# Autodesk Inventor assembly: Bartender Robot Asm
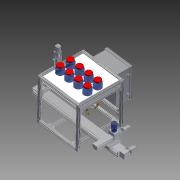
[picture p0: Inventor's stored thumbnail of the model, 180x180]
Saved by Autodesk Inventor 2011 (Build 150239000, 239)
## iProperties
Created: 2013-10-23
Part Number: Bartender Robot Asm
Document SubType Name: Assembly
Designer: Devon
Author: Devon
## Documents named in this file (31)
- C:\Users\Devon\Dropbox\ELEC 4497 - Senior Design\Design\Bartender Robot Asm.iam
- C:\Users\Devon\Dropbox\ELEC 4497 - Senior Design\Design\1.5 in. aluminum extrusion\Imported Components\47065T210\Part32.ipt
- C:\Users\Devon\Dropbox\ELEC 4497 - Senior Design\Design\1.5 in. aluminum extrusion\Imported Components\47065T210\Part34.ipt
- C:\Users\Devon\Dropbox\ELEC 4497 - Senior Design\Design\extrusion fittings\Imported Components\1.5in 3 sided fastener\Assembly5.iam
- C:\Users\Devon\Dropbox\ELEC 4497 - Senior Design\Design\extrusion fittings\Imported Components\1.5in 3 sided fastener\Assembly1.iam
- C:\Users\Devon\Dropbox\ELEC 4497 - Senior Design\Design\1.5 in. aluminum extrusion\Imported Components\47065T210\Part10.ipt
- C:\Users\Devon\Dropbox\ELEC 4497 - Senior Design\Design\extrusion fittings\Imported Components\1.5in 2 sided fastener\Assembly2.iam
- C:\Users\Devon\Dropbox\ELEC 4497 - Senior Design\Design\Enclosure\Imported Components\Enclosure\Assembly3.iam
- C:\Users\Devon\Dropbox\ELEC 4497 - Senior Design\Design\340mm KR linear actuator\PARTserver64610126with cover\KR45H 10A + 340L0 - 10A0(0-0).iam
- C:\Users\Devon\Dropbox\ELEC 4497 - Senior Design\Design\Liquid Vessel\Vessel.ipt
- C:\Users\Devon\Dropbox\ELEC 4497 - Senior Design\Design\1.5 in. aluminum extrusion\Imported Components\47065T210\Part3.ipt
- C:\Users\Devon\Dropbox\ELEC 4497 - Senior Design\Design\lexan panels\vessel support bottom.ipt
- C:\Users\Devon\Dropbox\ELEC 4497 - Senior Design\Design\lexan panels\vessel support top.ipt
- C:\Users\Devon\Dropbox\ELEC 4497 - Senior Design\Design\1.5 in. aluminum extrusion\Imported Components\47065T210\Part5.ipt
- C:\Users\Devon\Dropbox\ELEC 4497 - Senior Design\Design\machined mounts\xy axis mount.ipt
- C:\Users\Devon\Dropbox\ELEC 4497 - Senior Design\Design\machined mounts\glass socket.ipt
- C:\Users\Devon\Dropbox\ELEC 4497 - Senior Design\Design\glass\glass.ipt
- C:\Users\Devon\Dropbox\ELEC 4497 - Senior Design\Design\1.5 in. aluminum extrusion\7in.ipt
- C:\Users\Devon\Dropbox\ELEC 4497 - Senior Design\Design\servo motor\nema 23 frame size servo.ipt
- C:\Users\Devon\Dropbox\ELEC 4497 - Senior Design\Design\980mm KR linear actuator\NEMA23 frame size\GL20N-142-SW-EH--C-N-N-Y_(804U1).iam
- C:\Users\Devon\Dropbox\ELEC 4497 - Senior Design\Design\flow\flow meter solenoid asm.iam
- C:\Users\Devon\Dropbox\ELEC 4497 - Senior Design\Design\lexan panels\mixer support.ipt
- C:\Users\Devon\Dropbox\ELEC 4497 - Senior Design\Design\1.5 in. aluminum extrusion\5.094in.ipt
- C:\Users\Devon\Dropbox\ELEC 4497 - Senior Design\Design\Imported Components\5537T510\Part4.ipt
- C:\Users\Devon\Dropbox\ELEC 4497 - Senior Design\Design\Imported Components\5537T510\Part6.ipt
- C:\Users\Devon\Dropbox\ELEC 4497 - Senior Design\Design\Imported Components\5537T510\Part8.ipt
- C:\Users\Devon\Dropbox\ELEC 4497 - Senior Design\Design\Imported Components\5537T510\Part10.ipt
- C:\Users\Devon\Dropbox\ELEC 4497 - Senior Design\Design\Imported Components\5537T510\Part12.ipt
- C:\Users\Devon\Dropbox\ELEC 4497 - Senior Design\Design\Liquid Vessel\cap.ipt
- C:\Users\Devon\Dropbox\ELEC 4497 - Senior Design\Design\lexan panels\splash guard.ipt
- C:\Users\Devon\Dropbox\ELEC 4497 - Senior Design\Design\1.5 in. aluminum extrusion\Imported Components\47065T210\Part4.ipt
## Components (93 placed, 28 different names)
1. Part32:2 — Mate:10, Flush:19, Flush:20, Mate:15, Flush:27, Flush:28, Mate:30, Mate:103, Flush:92, Mate:106
2. Part32:3 — Mate:5, Flush:9, Flush:10, Mate:13, Flush:23, Flush:24, Flush:36, Flush:42, Mate:52, Mate:89, Flush:85, Mate:91, Flush:86, Mate:98, Flush:89, Mate:99, Flush:90, Flush:102, Mate:130, Flush:103, Mate:132, Flush:104
3. Part32:4 — Mate:2, Flush:3, Flush:4, Mate:9, Flush:17, Flush:18, Mate:125, Flush:111
4. Part32:5 — Mate:8, Flush:15, Flush:16, Mate:14, Flush:25, Flush:26, Flush:43, Mate:93, Flush:87, Mate:96, Flush:88, Mate:107, Mate:110
5. Part32:6 — Mate:1, Flush:1, Flush:2, Flush:3, Mate:4, Flush:7, Flush:8, Flush:55
6. Part32:7 — Mate:6, Flush:11, Flush:12, Mate:7, Flush:13, Flush:14, Mate:19, Flush:35
7. Part34:1 — Mate:3, Flush:5, Flush:6, Mate:16, Flush:29, Flush:30, Mate:29, Mate:101, Flush:91, Mate:112, Mate:126, Mate:128, Mate:134, Flush:105, Mate:136, Flush:106
8. Assembly5:1 [sub-assembly] — Mate:1, Flush:1, Flush:2, Mate:2, Flush:4, Mate:3, Flush:5, Flush:6
9. Assembly1:1 [sub-assembly] — Mate:4, Flush:7, Flush:8, Mate:5, Flush:9, Flush:10, Mate:6, Flush:11, Flush:12, Mate:21
10. Assembly1:2 [sub-assembly] — Mate:7, Flush:13, Flush:14, Mate:8, Flush:15, Flush:16, Mate:11, Flush:22
11. Assembly1:3 [sub-assembly] — Mate:9, Flush:17, Flush:18, Mate:10, Flush:19, Flush:20, Mate:12, Flush:21
12. Part10:1 — Mate:11, Mate:12, Flush:21, Flush:22, Mate:56
13. Part10:2 — Mate:17, Flush:31, Flush:32, Mate:73, Flush:77, Mate:75, Flush:78, Mate:86, Mate:87, Flush:84
14. Part10:3 — Mate:18, Flush:33, Flush:34, Mate:22, Flush:38, Mate:23, Flush:39, Mate:78, Mate:79, Flush:80, Mate:81, Flush:81, Mate:83, Flush:82
15. Assembly2:1 [sub-assembly] — Mate:16, Flush:29, Flush:30
16. Assembly2:2 [sub-assembly] — Mate:13, Flush:23, Flush:24, Mate:18, Flush:33, Flush:34, Mate:20
17. Assembly2:3 [sub-assembly] — Mate:14, Flush:25, Flush:26
18. Assembly2:4 [sub-assembly] — Mate:15, Flush:27, Flush:28, Mate:17, Flush:31, Flush:32
19. Assembly3:1 [sub-assembly] — Mate:19, Flush:35, Flush:37, Mate:21
20. Part32:8 — Mate:20, Flush:36, Flush:37, Mate:90, Mate:92, Mate:94, Mate:95
21. Part34:2 — Mate:22, Flush:38, Tangent:2, Tangent:5, Mate:46, Mate:82, Mate:84, Mate:85, Flush:83, Mate:88
22. Part34:3 — Mate:23, Flush:39, Tangent:3, Tangent:4, Mate:74, Mate:76, Mate:77, Flush:79, Mate:80
23. KR45H 10A + 340L0 - 10A0(0-0):1 [sub-assembly] — Flush:51, Flush:52, Mate:38, Flush:63, Mate:47, Flush:64, Flush:67, Flush:68, Mate:50
24. Vessel:1 — Insert:10, Mate:61, Mate:124, Insert:16
25. Vessel:2 — Insert:11, Mate:57, Mate:120, Insert:15
26. Part3:2 — Mate:29, Flush:42, Flush:59, Mate:55, Mate:97, Mate:100, Mate:102, Mate:111, Flush:96, Mate:139
27. vessel support bottom:1 — Insert:4, Insert:5, Insert:6, Insert:7, Insert:8, Insert:9, Insert:10, Insert:11, Mate:52, Mate:53, Mate:54, Mate:55, Tangent:6, Tangent:7, Tangent:8, Tangent:9, Tangent:10, Tangent:11, Tangent:12, Tangent:13, Flush:112, Flush:113, Flush:114, Flush:115, Flush:116, Flush:117, Flush:118, Flush:119
28. vessel support top:1 — Flush:55, Flush:59, Mate:56
29. Part5:2 — Mate:30, Flush:43, Mate:53, Mate:54, Mate:104, Mate:105, Flush:93, Mate:108, Flush:94, Mate:109, Flush:95
30. xy axis mount:1 — Flush:63, Mate:47, Flush:64, Mate:48, Flush:65, Flush:66
31. glass socket:1 — Flush:51, Flush:52, Mate:38, Insert:2
32. glass:1 — Insert:2
33. Vessel:3 — Insert:7, Mate:60, Mate:117, Insert:12
34. Vessel:4 — Insert:4, Mate:63, Mate:122, Insert:18
35. Vessel:5 — Insert:8, Mate:62, Mate:123, Insert:17
36. Vessel:6 — Insert:5, Mate:64, Mate:121, Insert:19
37. Vessel:7 — Insert:6, Mate:59, Mate:118, Insert:13
38. Vessel:8 — Insert:9, Mate:58, Mate:119, Insert:14
39. 7in:1 — Mate:65, Mate:67, Mate:69, Flush:71, Flush:72, Mate:114, Flush:101, Flush:108, Flush:109
40. 7in:2 — Mate:68, Mate:70, Flush:73, Flush:74, Mate:115, Flush:98, Mate:137, Mate:138, Flush:107
41. KR45H 10A + 340L0 - 10A0(0-0):2 [sub-assembly] — Flush:61, Flush:62, Mate:49, Flush:110, Mate:139
42. nema 23 frame size servo:1 — Flush:61, Flush:62, Mate:49
43. GL20N-142-SW-EH--C-N-N-Y_(804U1):1 [sub-assembly] — Tangent:2, Tangent:3, Tangent:4, Tangent:5, Mate:46, Mate:48, Flush:65, Flush:66, Flush:69, Flush:70, Mate:140
44. nema 23 frame size servo:2 — Flush:67, Flush:68, Mate:50
45. nema 23 frame size servo:3 — Flush:69, Flush:70, Mate:140
46. flow meter solenoid asm:1 [sub-assembly] — Mate:57, Tangent:6, Flush:119
47. flow meter solenoid asm:2 [sub-assembly] — Mate:63, Tangent:12, Flush:114
48. flow meter solenoid asm:3 [sub-assembly] — Mate:61, Tangent:10, Flush:112
49. flow meter solenoid asm:4 [sub-assembly] — Mate:64, Tangent:13, Flush:115
50. flow meter solenoid asm:5 [sub-assembly] — Mate:62, Tangent:11, Flush:113
51. flow meter solenoid asm:6 [sub-assembly] — Mate:58, Tangent:7, Flush:118
52. flow meter solenoid asm:7 [sub-assembly] — Mate:59, Tangent:8, Flush:117
53. flow meter solenoid asm:8 [sub-assembly] — Mate:60, Tangent:9, Flush:116
54. mixer support:1 — Mate:65, Mate:67, Mate:68, Mate:127
55. Assembly2:5 [sub-assembly] — Mate:69, Flush:71, Flush:72, Mate:72, Flush:75, Flush:76
56. Assembly2:6 [sub-assembly] — Mate:70, Flush:73, Flush:74, Mate:71, Flush:99, Flush:100
57. 5.094in:1 — Mate:71, Mate:72, Flush:75, Flush:76, Flush:99, Flush:100, Mate:127
58. Part4:1 — Mate:73, Mate:74, Flush:77
59. Part6:1 — Mate:77, Mate:78, Flush:79
60. Part6:2 — Mate:81, Mate:82, Flush:81
61. Part6:3 — Mate:75, Mate:76, Flush:78
62. Part6:4 — Mate:89, Mate:90, Flush:85
63. Part6:5 — Mate:93, Mate:94, Flush:87
64. Part6:6 — Mate:101, Mate:102, Flush:91
65. Part6:7 — Mate:87, Mate:88, Flush:84
66. Part6:8 — Mate:91, Mate:92, Flush:86
67. Part6:9 — Mate:85, Mate:86, Flush:83
68. Part6:10 — Mate:103, Mate:104, Flush:92
69. Part6:11 — Mate:105, Mate:106, Flush:93
70. Part6:12 — Mate:99, Mate:100, Flush:90
71. Part6:13 — Mate:97, Mate:98, Flush:89
72. Part6:14 — Mate:107, Mate:108, Flush:94
73. Part6:15 — Mate:83, Mate:84, Flush:82
74. Part6:16 — Mate:95, Mate:96, Flush:88
75. Part6:17 — Mate:79, Mate:80, Flush:80
76. Part8:1 — Mate:109, Mate:110, Flush:95
77. Part10:4 — Mate:111, Mate:112, Flush:96
78. Part12:1 — Mate:114, Flush:101, Flush:108
79. Part12:2 — Mate:115, Flush:98, Mate:138, Flush:107
80. cap:1 — Mate:122, Insert:18
81. cap:2 — Mate:123, Insert:17
82. cap:3 — Mate:124, Insert:16
83. cap:4 — Mate:121, Insert:19
84. cap:5 — Mate:120, Insert:15
85. cap:6 — Mate:119, Insert:14
86. cap:7 — Mate:118, Insert:13
87. cap:8 — Mate:117, Insert:12
88. splash guard:1 — Mate:125, Mate:126, Flush:111
89. Part4:2 — Mate:128, Flush:102, Mate:129, Mate:131, Mate:133, Mate:135, Mate:137, Flush:109, Flush:110
90. Part6:18 — Mate:131, Mate:132, Flush:104
91. Part6:19 — Mate:129, Mate:130, Flush:103
92. Part6:20 — Mate:133, Mate:134, Flush:105
93. Part6:21 — Mate:135, Mate:136, Flush:106
## Relationships (249: Mate 117, Flush 103, Insert 17, Tangent 12)
- Mate:1: Part32:6 ↔ Assembly5:1
- Flush:1 (12.2936 mm): Part32:6 ↔ Assembly5:1
- Flush:2 (12.2936 mm): Part32:6 ↔ Assembly5:1
- Mate:2: Part32:4 ↔ Assembly5:1
- Flush:3: Part32:4 ↔ Part32:6
- Flush:4 (12.2936 mm): Part32:4 ↔ Assembly5:1
- Mate:3: Part34:1 ↔ Assembly5:1
- Flush:5 (12.2936 mm): Part34:1 ↔ Assembly5:1
- Flush:6 (12.2936 mm): Part34:1 ↔ Assembly5:1
- Mate:4: Part32:6 ↔ Assembly1:1
- Flush:7 (12.2936 mm): Part32:6 ↔ Assembly1:1
- Flush:8 (12.2936 mm): Part32:6 ↔ Assembly1:1
- Mate:5: Part32:3 ↔ Assembly1:1
- Flush:9 (12.2936 mm): Part32:3 ↔ Assembly1:1
- Flush:10 (12.2936 mm): Part32:3 ↔ Assembly1:1
- Mate:6: Part32:7 ↔ Assembly1:1
- Flush:11 (12.2936 mm): Part32:7 ↔ Assembly1:1
- Flush:12 (12.2936 mm): Part32:7 ↔ Assembly1:1
- Mate:7: Part32:7 ↔ Assembly1:2
- Flush:13 (-12.2936 mm): Part32:7 ↔ Assembly1:2
- Flush:14 (-12.2936 mm): Part32:7 ↔ Assembly1:2
- Mate:8: Part32:5 ↔ Assembly1:2
- Flush:15 (12.2936 mm): Part32:5 ↔ Assembly1:2
- Flush:16 (12.2936 mm): Part32:5 ↔ Assembly1:2
- Mate:9: Part32:4 ↔ Assembly1:3
- Flush:17 (-12.2936 mm): Part32:4 ↔ Assembly1:3
- Flush:18 (-12.2936 mm): Part32:4 ↔ Assembly1:3
- Mate:10: Part32:2 ↔ Assembly1:3
- Flush:19 (12.2936 mm): Part32:2 ↔ Assembly1:3
- Flush:20 (12.2936 mm): Part32:2 ↔ Assembly1:3
- Mate:11: Assembly1:2 ↔ Part10:1
- Mate:12: Assembly1:3 ↔ Part10:1
- Flush:21 (12.2936 mm): Assembly1:3 ↔ Part10:1
- Flush:22 (12.2936 mm): Assembly1:2 ↔ Part10:1
- Mate:13: Part32:3 ↔ Assembly2:2
- Flush:23 (-12.2936 mm): Part32:3 ↔ Assembly2:2
- Flush:24 (-12.2936 mm): Part32:3 ↔ Assembly2:2
- Mate:14: Part32:5 ↔ Assembly2:3
- Flush:25 (-12.2936 mm): Part32:5 ↔ Assembly2:3
- Flush:26 (-12.2936 mm): Part32:5 ↔ Assembly2:3
- Mate:15: Part32:2 ↔ Assembly2:4
- Flush:27 (-12.2936 mm): Part32:2 ↔ Assembly2:4
- Flush:28 (-12.2936 mm): Part32:2 ↔ Assembly2:4
- Mate:16: Part34:1 ↔ Assembly2:1
- Flush:29 (-12.2936 mm): Part34:1 ↔ Assembly2:1
- Flush:30 (-12.2936 mm): Part34:1 ↔ Assembly2:1
- Mate:17: Part10:2 ↔ Assembly2:4
- Flush:31 (12.2936 mm): Part10:2 ↔ Assembly2:4
- Flush:32 (12.2936 mm): Part10:2 ↔ Assembly2:4
- Mate:18: Part10:3 ↔ Assembly2:2
- Flush:33 (12.2936 mm): Part10:3 ↔ Assembly2:2
- Flush:34 (12.2936 mm): Part10:3 ↔ Assembly2:2
- Mate:19 (12.2936 mm): Part32:7 ↔ Assembly3:1
- Flush:35 (-2.54 mm): Part32:7 ↔ Assembly3:1
- Mate:20: Assembly2:2 ↔ Part32:8
- Flush:36: Part32:3 ↔ Part32:8
- Flush:37 (2.54 mm): Assembly3:1 ↔ Part32:8
- Mate:21 (98.552 mm): Assembly1:1 ↔ Assembly3:1
- Mate:22 (12.2936 mm): Part10:3 ↔ Part34:2
- Flush:38: Part10:3 ↔ Part34:2
- Mate:23 (12.2936 mm): Part10:3 ↔ Part34:3
- Flush:39: Part10:3 ↔ Part34:3
- Mate:29 (12.2936 mm): Part34:1 ↔ Part3:2
- Flush:42: Part32:3 ↔ Part3:2
- Mate:30 (12.2936 mm): Part32:2 ↔ Part5:2
- Flush:43: Part32:5 ↔ Part5:2
- Flush:51: KR45H 10A + 340L0 - 10A0(0-0):1 ↔ glass socket:1
- Flush:52: KR45H 10A + 340L0 - 10A0(0-0):1 ↔ glass socket:1
- Mate:38: KR45H 10A + 340L0 - 10A0(0-0):1 ↔ glass socket:1
- Insert:2: glass socket:1 ↔ glass:1
- Insert:4 (6.35 mm): vessel support bottom:1 ↔ Vessel:4
- Insert:5 (6.35 mm): vessel support bottom:1 ↔ Vessel:6
- Insert:6 (6.35 mm): vessel support bottom:1 ↔ Vessel:7
- Insert:7 (6.35 mm): vessel support bottom:1 ↔ Vessel:3
- Insert:8 (6.35 mm): vessel support bottom:1 ↔ Vessel:5
- Insert:9 (6.35 mm): vessel support bottom:1 ↔ Vessel:8
- Insert:10 (6.35 mm): Vessel:1 ↔ vessel support bottom:1
- Insert:11 (6.35 mm): Vessel:2 ↔ vessel support bottom:1
- Flush:55 (12.2936 mm): Part32:6 ↔ vessel support top:1
- Flush:59: Part3:2 ↔ vessel support top:1
- Flush:61 (2.667 mm): KR45H 10A + 340L0 - 10A0(0-0):2 ↔ nema 23 frame size servo:1
- Flush:62 (1.4224 mm): KR45H 10A + 340L0 - 10A0(0-0):2 ↔ nema 23 frame size servo:1
- Tangent:2: Part34:2 ↔ GL20N-142-SW-EH--C-N-N-Y_(804U1):1
- Tangent:3: Part34:3 ↔ GL20N-142-SW-EH--C-N-N-Y_(804U1):1
- Tangent:4: Part34:3 ↔ GL20N-142-SW-EH--C-N-N-Y_(804U1):1
- Tangent:5: Part34:2 ↔ GL20N-142-SW-EH--C-N-N-Y_(804U1):1
- Mate:46 (12.2936 mm): Part34:2 ↔ GL20N-142-SW-EH--C-N-N-Y_(804U1):1
- Flush:63 (50.2031 mm): KR45H 10A + 340L0 - 10A0(0-0):1 ↔ xy axis mount:1
- Mate:47: KR45H 10A + 340L0 - 10A0(0-0):1 ↔ xy axis mount:1
- Flush:64 (141.8844 mm): KR45H 10A + 340L0 - 10A0(0-0):1 ↔ xy axis mount:1
- Mate:48: xy axis mount:1 ↔ GL20N-142-SW-EH--C-N-N-Y_(804U1):1
- Flush:65: xy axis mount:1 ↔ GL20N-142-SW-EH--C-N-N-Y_(804U1):1
- Flush:66: xy axis mount:1 ↔ GL20N-142-SW-EH--C-N-N-Y_(804U1):1
- Mate:49: KR45H 10A + 340L0 - 10A0(0-0):2 ↔ nema 23 frame size servo:1
- Flush:67 (2.667 mm): KR45H 10A + 340L0 - 10A0(0-0):1 ↔ nema 23 frame size servo:2
- Flush:68 (-1.4224 mm): KR45H 10A + 340L0 - 10A0(0-0):1 ↔ nema 23 frame size servo:2
- Mate:50: KR45H 10A + 340L0 - 10A0(0-0):1 ↔ nema 23 frame size servo:2
- Flush:69 (4.191 mm): GL20N-142-SW-EH--C-N-N-Y_(804U1):1 ↔ nema 23 frame size servo:3
- Flush:70 (4.445 mm): GL20N-142-SW-EH--C-N-N-Y_(804U1):1 ↔ nema 23 frame size servo:3
- Mate:52 (12.2936 mm): Part32:3 ↔ vessel support bottom:1
- Mate:53: vessel support bottom:1 ↔ Part5:2
- Mate:54: vessel support bottom:1 ↔ Part5:2
- Mate:55: Part3:2 ↔ vessel support bottom:1
- Mate:56: Part10:1 ↔ vessel support top:1
- Mate:57: Vessel:2 ↔ flow meter solenoid asm:1
- Tangent:6: vessel support bottom:1 ↔ flow meter solenoid asm:1
- Mate:58: Vessel:8 ↔ flow meter solenoid asm:6
- Tangent:7: vessel support bottom:1 ↔ flow meter solenoid asm:6
- Mate:59: Vessel:7 ↔ flow meter solenoid asm:7
- Tangent:8: vessel support bottom:1 ↔ flow meter solenoid asm:7
- Mate:60: Vessel:3 ↔ flow meter solenoid asm:8
- Tangent:9: vessel support bottom:1 ↔ flow meter solenoid asm:8
- Mate:61: Vessel:1 ↔ flow meter solenoid asm:3
- Tangent:10: vessel support bottom:1 ↔ flow meter solenoid asm:3
- Mate:62: Vessel:5 ↔ flow meter solenoid asm:5
- Tangent:11: vessel support bottom:1 ↔ flow meter solenoid asm:5
- Mate:63: Vessel:4 ↔ flow meter solenoid asm:2
- Tangent:12: vessel support bottom:1 ↔ flow meter solenoid asm:2
- Mate:64: Vessel:6 ↔ flow meter solenoid asm:4
- Tangent:13: vessel support bottom:1 ↔ flow meter solenoid asm:4
- Mate:65: 7in:1 ↔ mixer support:1
- Mate:67: 7in:1 ↔ mixer support:1
- Mate:68: 7in:2 ↔ mixer support:1
- Mate:69: 7in:1 ↔ Assembly2:5
- Flush:71 (-12.2936 mm): 7in:1 ↔ Assembly2:5
- Flush:72 (-12.2936 mm): 7in:1 ↔ Assembly2:5
- Mate:70: 7in:2 ↔ Assembly2:6
- Flush:73 (-12.2936 mm): 7in:2 ↔ Assembly2:6
- Flush:74 (-12.2936 mm): 7in:2 ↔ Assembly2:6
- Mate:71: Assembly2:6 ↔ 5.094in:1
- Mate:72: Assembly2:5 ↔ 5.094in:1
- Flush:75 (12.2936 mm): Assembly2:5 ↔ 5.094in:1
- Flush:76 (12.2936 mm): Assembly2:5 ↔ 5.094in:1
- Mate:73 (12.2936 mm): Part10:2 ↔ Part4:1
- Mate:74 (12.2936 mm): Part34:3 ↔ Part4:1
- Flush:77 (-12.2936 mm): Part10:2 ↔ Part4:1
- Mate:75 (12.2936 mm): Part10:2 ↔ Part6:3
- Mate:76 (12.2936 mm): Part34:3 ↔ Part6:3
- Flush:78 (-12.2936 mm): Part10:2 ↔ Part6:3
- Mate:77 (12.2936 mm): Part34:3 ↔ Part6:1
- Mate:78 (12.2936 mm): Part10:3 ↔ Part6:1
- Flush:79 (-12.2936 mm): Part34:3 ↔ Part6:1
- Mate:79 (12.2936 mm): Part10:3 ↔ Part6:17
- Mate:80 (12.2936 mm): Part34:3 ↔ Part6:17
- Flush:80 (-12.2936 mm): Part10:3 ↔ Part6:17
- Mate:81 (12.2936 mm): Part10:3 ↔ Part6:2
- Mate:82 (12.2936 mm): Part34:2 ↔ Part6:2
- Flush:81 (-12.2936 mm): Part10:3 ↔ Part6:2
- Mate:83 (12.2936 mm): Part10:3 ↔ Part6:15
- Mate:84 (12.2936 mm): Part34:2 ↔ Part6:15
- Flush:82 (-12.2936 mm): Part10:3 ↔ Part6:15
- Mate:85 (12.2936 mm): Part34:2 ↔ Part6:9
- Mate:86 (12.2936 mm): Part10:2 ↔ Part6:9
- Flush:83 (-12.2936 mm): Part34:2 ↔ Part6:9
- Mate:87 (12.2936 mm): Part10:2 ↔ Part6:7
- Mate:88 (12.2936 mm): Part34:2 ↔ Part6:7
- Flush:84 (-12.2936 mm): Part10:2 ↔ Part6:7
- Mate:89 (12.2936 mm): Part32:3 ↔ Part6:4
- Mate:90 (12.2936 mm): Part32:8 ↔ Part6:4
- Flush:85 (-12.2936 mm): Part32:3 ↔ Part6:4
- Mate:91 (12.2936 mm): Part32:3 ↔ Part6:8
- Mate:92 (12.2936 mm): Part32:8 ↔ Part6:8
- Flush:86 (-12.2936 mm): Part32:3 ↔ Part6:8
- Mate:93 (12.2936 mm): Part32:5 ↔ Part6:5
- Mate:94 (12.2936 mm): Part32:8 ↔ Part6:5
- Flush:87 (-12.2936 mm): Part32:5 ↔ Part6:5
- Mate:95 (12.2936 mm): Part32:8 ↔ Part6:16
- Mate:96 (12.2936 mm): Part32:5 ↔ Part6:16
- Flush:88 (-12.2936 mm): Part32:5 ↔ Part6:16
- Mate:97 (12.2936 mm): Part3:2 ↔ Part6:13
- Mate:98 (12.2936 mm): Part32:3 ↔ Part6:13
- Flush:89 (-12.2936 mm): Part32:3 ↔ Part6:13
- Mate:99 (12.2936 mm): Part32:3 ↔ Part6:12
- Mate:100 (12.2936 mm): Part3:2 ↔ Part6:12
- Flush:90 (-12.2936 mm): Part32:3 ↔ Part6:12
- Mate:101 (12.2936 mm): Part34:1 ↔ Part6:6
- Mate:102 (12.2936 mm): Part3:2 ↔ Part6:6
- Flush:91 (-12.2936 mm): Part34:1 ↔ Part6:6
- Mate:103 (12.2936 mm): Part32:2 ↔ Part6:10
- Mate:104 (12.2936 mm): Part5:2 ↔ Part6:10
- Flush:92 (-12.2936 mm): Part32:2 ↔ Part6:10
- Mate:105 (12.2936 mm): Part5:2 ↔ Part6:11
- Mate:106 (12.2936 mm): Part32:2 ↔ Part6:11
- Flush:93 (-12.2936 mm): Part5:2 ↔ Part6:11
- Mate:107 (12.2936 mm): Part32:5 ↔ Part6:14
- Mate:108 (12.2936 mm): Part5:2 ↔ Part6:14
- Flush:94 (-12.2936 mm): Part5:2 ↔ Part6:14
- Mate:109 (12.2936 mm): Part5:2 ↔ Part8:1
- Mate:110 (12.2936 mm): Part32:5 ↔ Part8:1
- Flush:95 (-12.2936 mm): Part5:2 ↔ Part8:1
- Mate:111 (12.2936 mm): Part3:2 ↔ Part10:4
- Mate:112 (12.2936 mm): Part34:1 ↔ Part10:4
- Flush:96 (-12.2936 mm): Part3:2 ↔ Part10:4
- Mate:114 (12.2936 mm): 7in:1 ↔ Part12:1
- Mate:115 (12.2936 mm): 7in:2 ↔ Part12:2
- Flush:98 (-12.2936 mm): 7in:2 ↔ Part12:2
- Mate:117: Vessel:3 ↔ cap:8
- Mate:118: Vessel:7 ↔ cap:7
- Mate:119: Vessel:8 ↔ cap:6
- Mate:120: Vessel:2 ↔ cap:5
- Mate:121: Vessel:6 ↔ cap:4
- Mate:122: Vessel:4 ↔ cap:1
- Mate:123: Vessel:5 ↔ cap:2
- Mate:124: Vessel:1 ↔ cap:3
- Insert:12: Vessel:3 ↔ cap:8
- Insert:13: Vessel:7 ↔ cap:7
- Insert:14: Vessel:8 ↔ cap:6
- Insert:15: Vessel:2 ↔ cap:5
- Insert:16: Vessel:1 ↔ cap:3
- Insert:17: Vessel:5 ↔ cap:2
- Insert:18: Vessel:4 ↔ cap:1
- Insert:19: Vessel:6 ↔ cap:4
- Mate:125: Part32:4 ↔ splash guard:1
- Mate:126: Part34:1 ↔ splash guard:1
- Flush:99 (-12.2936 mm): Assembly2:6 ↔ 5.094in:1
- Flush:100 (-12.2936 mm): Assembly2:6 ↔ 5.094in:1
- Flush:101: 7in:1 ↔ Part12:1
- Mate:127: mixer support:1 ↔ 5.094in:1
- Mate:128 (12.2936 mm): Part34:1 ↔ Part4:2
- Flush:102: Part32:3 ↔ Part4:2
- Mate:129 (12.2936 mm): Part4:2 ↔ Part6:19
- Mate:130 (12.2936 mm): Part32:3 ↔ Part6:19
- Flush:103 (-12.2936 mm): Part32:3 ↔ Part6:19
- Mate:131 (12.2936 mm): Part4:2 ↔ Part6:18
- Mate:132 (12.2936 mm): Part32:3 ↔ Part6:18
- Flush:104 (-12.2936 mm): Part32:3 ↔ Part6:18
- Mate:133 (12.2936 mm): Part4:2 ↔ Part6:20
- Mate:134 (12.2936 mm): Part34:1 ↔ Part6:20
- Flush:105 (-12.2936 mm): Part34:1 ↔ Part6:20
- Mate:135 (12.2936 mm): Part4:2 ↔ Part6:21
- Mate:136 (12.2936 mm): Part34:1 ↔ Part6:21
- Flush:106 (-12.2936 mm): Part34:1 ↔ Part6:21
- Mate:137 (12.2936 mm): 7in:2 ↔ Part4:2
- Mate:138 (12.2936 mm): 7in:2 ↔ Part12:2
- Flush:107: 7in:2 ↔ Part12:2
- Flush:108 (-12.2936 mm): 7in:1 ↔ Part12:1
- Flush:109: 7in:1 ↔ Part4:2
- Flush:110 (-12.2936 mm): KR45H 10A + 340L0 - 10A0(0-0):2 ↔ Part4:2
- Mate:139 (12.2936 mm): Part3:2 ↔ KR45H 10A + 340L0 - 10A0(0-0):2
- Flush:111: Part32:4 ↔ splash guard:1
- Flush:112 (-207.772 mm): vessel support bottom:1 ↔ flow meter solenoid asm:3
- Flush:113 (-207.772 mm): vessel support bottom:1 ↔ flow meter solenoid asm:5
- Flush:114 (-207.772 mm): vessel support bottom:1 ↔ flow meter solenoid asm:2
- Flush:115 (-207.772 mm): vessel support bottom:1 ↔ flow meter solenoid asm:4
- Flush:116 (-207.772 mm): vessel support bottom:1 ↔ flow meter solenoid asm:8
- Flush:117 (-207.772 mm): vessel support bottom:1 ↔ flow meter solenoid asm:7
- Flush:118 (-207.7212 mm): vessel support bottom:1 ↔ flow meter solenoid asm:6
- Flush:119 (-207.5942 mm): vessel support bottom:1 ↔ flow meter solenoid asm:1
- Mate:140: GL20N-142-SW-EH--C-N-N-Y_(804U1):1 ↔ nema 23 frame size servo:3
